# Autodesk Inventor assembly: RoundPhantomAssembly_01Nov20
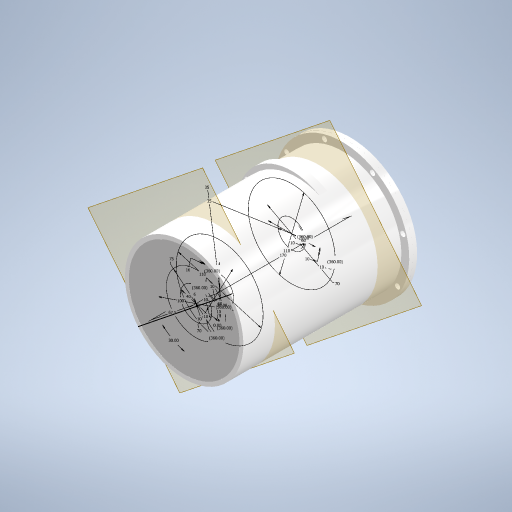
[picture p0: Inventor's stored thumbnail of the model, 512x512]
Saved by Autodesk Inventor 2024.2 (Build 282272000, 272)
## iProperties
Created: 2020-11-02
Part Number: RoundPhantomAssembly_01Nov20
Document SubType Name: Assembly
Designer: uqphoop1
Author: uqphoop1
## iProperties of the stored document MemberDocs/xAaaaqbcaAaaaaaaaAaaaqxjcCb
Created: 2020-11-02
Part Number: RoundPhantomAssembly_01Nov20
Document SubType Name: Assembly
Designer: uqphoop1
Author: uqphoop1
## Documents named in this file (12)
- Z:\Phantom-Design-Files\RoundPhantomAssembly_Final.iam
- Z:\Phantom-Design-Files\input-files\Flange Base_Final.ipt
- Z:\Phantom-Design-Files\input-files\Flange Top_Final.ipt
- Z:\Phantom-Design-Files\input-files\Medium Tube + Medium Cap.iam
- Z:\Phantom-Design-Files\input-files\Main Outer Part - 140 (ID), 150 (OD)_Final.ipt
- Z:\Phantom-Design-Files\input-files\Bottom Plate_Final.ipt
- Z:\Phantom-Design-Files\input-files\Small Tube_forMainAssembly.ipt
- Z:\Phantom-Design-Files\input-files\Large tube_forMainAssembly.ipt
- Z:\Phantom-Design-Files\input-files\Supporting Plate_Final.ipt
- Z:\Phantom-Design-Files\RoundPhantomAssembly_Final\Design Accelerator\O-Ring1.iam
- C:\Users\s4601543\OneDrive - The University of Queensland\Documents\Inventor\Content Center Files\R2024\en-US\Nylon BS 4183 Slotted Cheese Head Machine Screw - Metric M12 x 16\M12 x 16-Nylon 6_6.ipt
- C:\Users\s4601543\OneDrive - The University of Queensland\Documents\Inventor\Content Center Files\R2024\en-US\Nylon BS 4183 Slotted Cheese Head Machine Screw - Metric M6 x 16\M6 x 16-6.ipt
## Components (25 placed, 8 different names)
1. Flange Base_Final:1 — Insert:1, Insert:2, Insert:11, Mate:46, Insert:35, Mate:57, Mate:61, Insert:39
2. Flange Top_Final:1 — Insert:1, Insert:2, Mate:61
3. Medium Tube + Medium Cap:1 [sub-assembly] — Mate:48, Insert:40
4. Main Outer Part - 140 (ID), 150 (OD)_Final:1 — Insert:11, Insert:36, Insert:37, Mate:63
5. Bottom Plate_Final:1 — Insert:14, Insert:15, Insert:16, Insert:17, Insert:18, Insert:19, Insert:27, Insert:28, Insert:29, Insert:30, Insert:31, Insert:32, Insert:35, Mate:56, Mate:57, Mate:63, Insert:40, Mate:64, Mate:65, Mate:66, Mate:67, Mate:68, Mate:69
6. Small Tube_forMainAssembly:1 — Insert:14
7. Small Tube_forMainAssembly:2 — Insert:15
8. Small Tube_forMainAssembly:3 — Insert:16
9. Small Tube_forMainAssembly:4 — Insert:17
10. Small Tube_forMainAssembly:5 — Insert:19
11. Small Tube_forMainAssembly:6 — Insert:18
12. Medium Tube + Medium Cap:2 [sub-assembly] — Mate:68
13. Medium Tube + Medium Cap:3 [sub-assembly] — Mate:67
14. Medium Tube + Medium Cap:4 [sub-assembly] — Mate:66
15. Medium Tube + Medium Cap:5 [sub-assembly] — Mate:65
16. Medium Tube + Medium Cap:6 [sub-assembly] — Mate:64
17. Medium Tube + Medium Cap:7 [sub-assembly] — Mate:69
18. Large tube_forMainAssembly:1 — Insert:28
19. Large tube_forMainAssembly:2 — Insert:29
20. Large tube_forMainAssembly:3 — Insert:32, Mate:46
21. Large tube_forMainAssembly:4 — Insert:27
22. Large tube_forMainAssembly:5 — Insert:31
23. Large tube_forMainAssembly:6 — Insert:30, Mate:62
24. Supporting Plate_Final:1 — Insert:36, Insert:37
25. Supporting Plate_Final:2 — Insert:39, Mate:62
## Relationships (33: Insert 20, Mate 13)
- Insert:1: Flange Base_Final:1 ↔ Flange Top_Final:1
- Insert:2: Flange Base_Final:1 ↔ Flange Top_Final:1
- Insert:11: Flange Base_Final:1 ↔ Main Outer Part - 140 (ID), 150 (OD)_Final:1
- Insert:14: Bottom Plate_Final:1 ↔ Small Tube_forMainAssembly:1
- Insert:15: Bottom Plate_Final:1 ↔ Small Tube_forMainAssembly:2
- Insert:16: Bottom Plate_Final:1 ↔ Small Tube_forMainAssembly:3
- Insert:17: Bottom Plate_Final:1 ↔ Small Tube_forMainAssembly:4
- Insert:18: Bottom Plate_Final:1 ↔ Small Tube_forMainAssembly:6
- Insert:19: Bottom Plate_Final:1 ↔ Small Tube_forMainAssembly:5
- Insert:27: Bottom Plate_Final:1 ↔ Large tube_forMainAssembly:4
- Insert:28: Bottom Plate_Final:1 ↔ Large tube_forMainAssembly:1
- Insert:29: Bottom Plate_Final:1 ↔ Large tube_forMainAssembly:2
- Insert:30: Bottom Plate_Final:1 ↔ Large tube_forMainAssembly:6
- Insert:31: Bottom Plate_Final:1 ↔ Large tube_forMainAssembly:5
- Insert:32: Bottom Plate_Final:1 ↔ Large tube_forMainAssembly:3
- Mate:46: Flange Base_Final:1 ↔ Large tube_forMainAssembly:3
- Insert:35 (180 mm): Flange Base_Final:1 ↔ Bottom Plate_Final:1
- Mate:48: Medium Tube + Medium Cap:1
- Mate:56: Bottom Plate_Final:1
- Mate:57 (180 mm): Flange Base_Final:1 ↔ Bottom Plate_Final:1
- Insert:36: Main Outer Part - 140 (ID), 150 (OD)_Final:1 ↔ Supporting Plate_Final:1
- Insert:37: Main Outer Part - 140 (ID), 150 (OD)_Final:1 ↔ Supporting Plate_Final:1
- Mate:61: Flange Base_Final:1 ↔ Flange Top_Final:1
- Insert:39 (20 mm): Flange Base_Final:1 ↔ Supporting Plate_Final:2
- Mate:62: Large tube_forMainAssembly:6 ↔ Supporting Plate_Final:2
- Mate:63: Main Outer Part - 140 (ID), 150 (OD)_Final:1 ↔ Bottom Plate_Final:1
- Insert:40: Medium Tube + Medium Cap:1 ↔ Bottom Plate_Final:1
- Mate:64: Bottom Plate_Final:1 ↔ Medium Tube + Medium Cap:6
- Mate:65: Bottom Plate_Final:1 ↔ Medium Tube + Medium Cap:5
- Mate:66: Bottom Plate_Final:1 ↔ Medium Tube + Medium Cap:4
- Mate:67: Bottom Plate_Final:1 ↔ Medium Tube + Medium Cap:3
- Mate:68: Bottom Plate_Final:1 ↔ Medium Tube + Medium Cap:2
- Mate:69: Bottom Plate_Final:1 ↔ Medium Tube + Medium Cap:7
